# Autodesk Inventor assembly: Scissor Lift
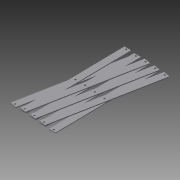
[picture p0: Inventor's stored thumbnail of the model, 180x180]
Saved by Autodesk Inventor 2015 (Build 190159000, 159)
## iProperties
Created: 2017-01-05
Part Number: Scissor Lift
Document SubType Name: Assembly
Designer: ps2du
Author: ps2du
## Documents named in this file (2)
- E:\Robo Parts Inventor\Scissor Lift.iam
- E:\Robo Parts Inventor\Jack FlatStock.ipt
## Components (8 placed, 1 different names)
1. Jack FlatStock:6 — Rotational:2, Rotational:4, Rotational:6
2. Jack FlatStock:7 — Rotational:2, Rotational:1, Rotational:7
3. Jack FlatStock:9 — Rotational:1, Rotational:5
4. Jack FlatStock:10 — Rotational:4, Rotational:5
5. Jack FlatStock:11 — Rotational:7, Rotational:8, Rotational:9
6. Jack FlatStock:12 — Rotational:6, Rotational:8, Rotational:10
7. Jack FlatStock:13 — Rotational:10, Rotational:11
8. Jack FlatStock:14 — Rotational:9, Rotational:11
## Relationships (10: RevoluteJoint 10)
- Rotational:2 [RevoluteJoint]: Jack FlatStock:6 ↔ Jack FlatStock:7
- Rotational:1 [RevoluteJoint]: Jack FlatStock:7 ↔ Jack FlatStock:9
- Rotational:4 [RevoluteJoint]: Jack FlatStock:6 ↔ Jack FlatStock:10
- Rotational:5 [RevoluteJoint]: Jack FlatStock:9 ↔ Jack FlatStock:10
- Rotational:6 [RevoluteJoint]: Jack FlatStock:6 ↔ Jack FlatStock:12
- Rotational:7 [RevoluteJoint]: Jack FlatStock:7 ↔ Jack FlatStock:11
- Rotational:8 [RevoluteJoint]: Jack FlatStock:11 ↔ Jack FlatStock:12
- Rotational:9 [RevoluteJoint]: Jack FlatStock:11 ↔ Jack FlatStock:14
- Rotational:10 [RevoluteJoint]: Jack FlatStock:12 ↔ Jack FlatStock:13
- Rotational:11 [RevoluteJoint]: Jack FlatStock:13 ↔ Jack FlatStock:14
